# Autodesk Inventor assembly: 200-20-ROCKER-CONNECTOR-ASM-01
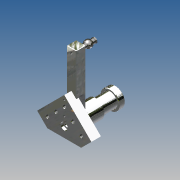
[picture p0: Inventor's stored thumbnail of the model, 180x180]
Saved by Autodesk Inventor 2018.2 (Build 222227000, 227)
## iProperties
Manager: feesmrt
Company: FRANC0R
Created: 2017-11-01
Part Number: 200-20-ROCKER-CONNECTOR-ASM-01
Material: Generisch
Document SubType Name: Assembly
Designer: feesmrt
Project: Rescue Robot
Cost Center: -
Description: Rocker Bearing Connector
Engineer: feesmrt
Authority: feesmrt
Stock Number: 200-20-ROCKER-CONNECTOR-ASM-01
Mass: 342.249 g
Surface Area: 374.371 cm^2
Volume: 115.439 cm^3
Density: 2.96477 g/cm^3
Author: feesmrt
Title: Rocker Bearing Connector
Subject: Rescue Robot
Revision Number: 1
## Documents named in this file (11)
- D:\Programmierung\FRANC0R\CAD\02-Rocker-Bogie-Robot\200-ROCKER-BOGIE\200-20-ROCKER-CONNECTOR\200-20-ROCKER-CONNECTOR-ASM-01.iam
- D:\Programmierung\FRANC0R\CAD\02-Rocker-Bogie-Robot\200-ROCKER-BOGIE\200-20-ROCKER-CONNECTOR\200-20-ROCKER-CONNECTOR-01.ipt
- D:\Programmierung\FRANC0R\CAD\02-Rocker-Bogie-Robot\200-ROCKER-BOGIE\200-20-ROCKER-CONNECTOR\200-20-ROCKER-CONNECTOR-02.ipt
- D:\Programmierung\FRANC0R\CAD\02-Rocker-Bogie-Robot\900-COMPONENTS\900-40-SCREWS\900-40-SCREWS-ISO10642_M6x16.ipt
- D:\Programmierung\FRANC0R\CAD\02-Rocker-Bogie-Robot\200-ROCKER-BOGIE\200-20-ROCKER-CONNECTOR\200-20-ROCKER-CONNECTOR-04.ipt
- D:\Programmierung\FRANC0R\CAD\02-Rocker-Bogie-Robot\900-COMPONENTS\900-40-SCREWS\900-40-SCREWS-DIN7984_M5x25.ipt
- D:\Programmierung\FRANC0R\CAD\02-Rocker-Bogie-Robot\200-ROCKER-BOGIE\200-60-DIFFERENTIAL\200-60-DIFFERENTIAL-BAR-01.ipt
- D:\Programmierung\FRANC0R\CAD\02-Rocker-Bogie-Robot\200-ROCKER-BOGIE\200-60-DIFFERENTIAL\200-60-DIFFERENTIAL-BAR-02.ipt
- D:\Programmierung\FRANC0R\CAD\02-Rocker-Bogie-Robot\900-COMPONENTS\900-41-NUTS\900-41-NUTS-ISO4035-M6.ipt
- D:\Programmierung\FRANC0R\CAD\02-Rocker-Bogie-Robot\900-COMPONENTS\900-70-ANGLE-JOINTS\900-70-ANGLE-JOINT-DIN648-M8-2.ipt
- D:\Programmierung\FRANC0R\CAD\02-Rocker-Bogie-Robot\200-ROCKER-BOGIE\200-60-DIFFERENTIAL\200-60-DIFFERENTIAL-BAR-04.ipt
## Components (12 placed, 10 different names)
1. 200-20-ROCKER-CONNECTOR-01:1 — Passend:1, Passend:2, Passend:29, Passend:30, Passend:31, Passend:33
2. 200-20-ROCKER-CONNECTOR-02:1 — Passend:1, Passend:2, Passend:4, Fluchtend:1
3. 900-40-SCREWS-ISO10642_M6x16:1 — Passend:4, Fluchtend:1
4. 200-20-ROCKER-CONNECTOR-04:1 — Passend:29, Passend:30, Passend:31, Passend:32, Passend:34
5. 900-40-SCREWS-DIN7984_M5x25:1 — Passend:35, Passend:37
6. 900-40-SCREWS-DIN7984_M5x25:2 — Passend:36, Passend:38
7. 200-60-DIFFERENTIAL-BAR-01:1 — Passend:32, Passend:33, Passend:34, Passend:35, Passend:36, Passend:37, Passend:38, Passend:39, Passend:42
8. 200-60-DIFFERENTIAL-BAR-02:1 — Passend:39, Passend:40, Passend:41, Passend:43, Passend:44, Passend:45, Passend:47
9. 900-41-NUTS-ISO4035-M6:1 — Passend:40, Passend:41, Passend:42
10. 900-70-ANGLE-JOINT-DIN648-M8-2:1 — Passend:43, Passend:44, Passend:46
11. 200-60-DIFFERENTIAL-BAR-04:1 — Passend:45, Passend:46, Passend:48
12. 900-41-NUTS-ISO4035-M6:2 — Passend:47, Passend:48
## Relationships (24: Mate 23, Flush 1)
- Passend:1 [Mate]: 200-20-ROCKER-CONNECTOR-01:1 ↔ 200-20-ROCKER-CONNECTOR-02:1
- Passend:2 [Mate]: 200-20-ROCKER-CONNECTOR-01:1 ↔ 200-20-ROCKER-CONNECTOR-02:1
- Passend:4 [Mate]: 200-20-ROCKER-CONNECTOR-02:1 ↔ 900-40-SCREWS-ISO10642_M6x16:1
- Fluchtend:1 [Flush]: 200-20-ROCKER-CONNECTOR-02:1 ↔ 900-40-SCREWS-ISO10642_M6x16:1
- Passend:29 [Mate]: 200-20-ROCKER-CONNECTOR-01:1 ↔ 200-20-ROCKER-CONNECTOR-04:1
- Passend:30 [Mate]: 200-20-ROCKER-CONNECTOR-01:1 ↔ 200-20-ROCKER-CONNECTOR-04:1
- Passend:31 [Mate]: 200-20-ROCKER-CONNECTOR-01:1 ↔ 200-20-ROCKER-CONNECTOR-04:1
- Passend:32 [Mate]: 200-20-ROCKER-CONNECTOR-04:1 ↔ 200-60-DIFFERENTIAL-BAR-01:1
- Passend:33 [Mate]: 200-20-ROCKER-CONNECTOR-01:1 ↔ 200-60-DIFFERENTIAL-BAR-01:1
- Passend:34 [Mate]: 200-20-ROCKER-CONNECTOR-04:1 ↔ 200-60-DIFFERENTIAL-BAR-01:1
- Passend:35 [Mate]: 900-40-SCREWS-DIN7984_M5x25:1 ↔ 200-60-DIFFERENTIAL-BAR-01:1
- Passend:36 [Mate]: 900-40-SCREWS-DIN7984_M5x25:2 ↔ 200-60-DIFFERENTIAL-BAR-01:1
- Passend:37 [Mate]: 900-40-SCREWS-DIN7984_M5x25:1 ↔ 200-60-DIFFERENTIAL-BAR-01:1
- Passend:38 [Mate]: 900-40-SCREWS-DIN7984_M5x25:2 ↔ 200-60-DIFFERENTIAL-BAR-01:1
- Passend:39 [Mate]: 200-60-DIFFERENTIAL-BAR-01:1 ↔ 200-60-DIFFERENTIAL-BAR-02:1
- Passend:40 [Mate]: 200-60-DIFFERENTIAL-BAR-02:1 ↔ 900-41-NUTS-ISO4035-M6:1
- Passend:41 [Mate] (0.602 mm): 200-60-DIFFERENTIAL-BAR-02:1 ↔ 900-41-NUTS-ISO4035-M6:1
- Passend:42 [Mate]: 200-60-DIFFERENTIAL-BAR-01:1 ↔ 900-41-NUTS-ISO4035-M6:1
- Passend:43 [Mate]: 200-60-DIFFERENTIAL-BAR-02:1 ↔ 900-70-ANGLE-JOINT-DIN648-M8-2:1
- Passend:44 [Mate]: 200-60-DIFFERENTIAL-BAR-02:1 ↔ 900-70-ANGLE-JOINT-DIN648-M8-2:1
- Passend:45 [Mate]: 200-60-DIFFERENTIAL-BAR-02:1 ↔ 200-60-DIFFERENTIAL-BAR-04:1
- Passend:46 [Mate]: 900-70-ANGLE-JOINT-DIN648-M8-2:1 ↔ 200-60-DIFFERENTIAL-BAR-04:1
- Passend:47 [Mate]: 200-60-DIFFERENTIAL-BAR-02:1 ↔ 900-41-NUTS-ISO4035-M6:2
- Passend:48 [Mate]: 200-60-DIFFERENTIAL-BAR-04:1 ↔ 900-41-NUTS-ISO4035-M6:2
